# Autodesk Inventor assembly: Stewart Assembly
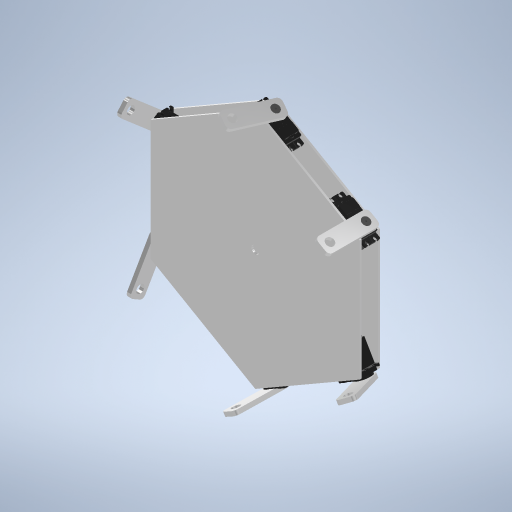
[picture p0: Inventor's stored thumbnail of the model, 512x512]
Saved by Autodesk Inventor 2023 (Build 270158000, 158)
## iProperties
Created: 2022-06-23
Part Number: Stewart Assembly
Document SubType Name: Assembly
Designer: earls
Mass: 1362.34 g
Surface Area: 2982.25 cm^2
Volume: 504.572 cm^3
Density: 2.7 g/cm^3
Author: earls
## Documents named in this file (4)
- F:\Documents\Mechatronic Engineering 5.1\Project\CAD\Stewart Assembly.iam
- F:\Documents\Mechatronic Engineering 5.1\Project\CAD\Bottom plate 2.5mm.ipt
- F:\Documents\Mechatronic Engineering 5.1\Project\CAD\ServoMotor\Servo.ipt
- F:\Documents\Mechatronic Engineering 5.1\Project\CAD\Servo arm.ipt
## Components (14 placed, 3 different names)
1. Bottom plate 2.5mm:1 — Mate:4, Mate:5, Mate:6, Mate:10, Mate:11, Mate:12, Mate:13, Mate:14, Mate:15, Mate:16, Mate:17, Mate:18, Mate:19, Mate:20, Mate:21, Mate:23, Mate:24, Mate:25, Mate:26, Mate:27, Mate:28, Mate:29, Mate:30
2. Servo:2 — Mate:4, Mate:5, Mate:6, Rotational:5
3. Servo:3 — Mate:28, Mate:29, Mate:30, Rotational:6
4. Servo:4 — Mate:10, Mate:11, Mate:12, Rotational:7
5. Servo:5 — Mate:13, Mate:14, Mate:15, Rotational:8
6. Servo:6 — Mate:16, Mate:17, Mate:18, Rotational:4
7. Servo:7 — Mate:19, Mate:20, Mate:21, Mate:22, Rotational:9
8. Bottom plate 2.5mm:2 — Mate:22, Mate:23, Mate:24, Mate:25, Mate:26, Mate:27
9. Servo arm:1 — Rotational:8
10. Servo arm:2 — Rotational:7
11. Servo arm:3 — Rotational:4
12. Servo arm:4 — Rotational:9
13. Servo arm:5 — Rotational:5
14. Servo arm:6 — Rotational:6
## Relationships (30: Mate 24, RevoluteJoint 6)
- Mate:4: Bottom plate 2.5mm:1 ↔ Servo:2
- Mate:5: Bottom plate 2.5mm:1 ↔ Servo:2
- Mate:6: Bottom plate 2.5mm:1 ↔ Servo:2
- Mate:10: Bottom plate 2.5mm:1 ↔ Servo:4
- Mate:11: Bottom plate 2.5mm:1 ↔ Servo:4
- Mate:12: Bottom plate 2.5mm:1 ↔ Servo:4
- Mate:13: Bottom plate 2.5mm:1 ↔ Servo:5
- Mate:14: Bottom plate 2.5mm:1 ↔ Servo:5
- Mate:15: Bottom plate 2.5mm:1 ↔ Servo:5
- Mate:16: Bottom plate 2.5mm:1 ↔ Servo:6
- Mate:17: Bottom plate 2.5mm:1 ↔ Servo:6
- Mate:18: Bottom plate 2.5mm:1 ↔ Servo:6
- Mate:19: Bottom plate 2.5mm:1 ↔ Servo:7
- Mate:20: Bottom plate 2.5mm:1 ↔ Servo:7
- Mate:21: Bottom plate 2.5mm:1 ↔ Servo:7
- Mate:22: Servo:7 ↔ Bottom plate 2.5mm:2
- Mate:23: Bottom plate 2.5mm:1 ↔ Bottom plate 2.5mm:2
- Mate:24: Bottom plate 2.5mm:1 ↔ Bottom plate 2.5mm:2
- Mate:25: Bottom plate 2.5mm:1 ↔ Bottom plate 2.5mm:2
- Mate:26: Bottom plate 2.5mm:1 ↔ Bottom plate 2.5mm:2
- Mate:27: Bottom plate 2.5mm:1 ↔ Bottom plate 2.5mm:2
- Rotational:4 [RevoluteJoint]: Servo:6 ↔ Servo arm:3
- Rotational:5 [RevoluteJoint]: Servo:2 ↔ Servo arm:5
- Mate:28: Bottom plate 2.5mm:1 ↔ Servo:3
- Mate:29: Bottom plate 2.5mm:1 ↔ Servo:3
- Mate:30: Bottom plate 2.5mm:1 ↔ Servo:3
- Rotational:6 [RevoluteJoint]: Servo:3 ↔ Servo arm:6
- Rotational:7 [RevoluteJoint]: Servo:4 ↔ Servo arm:2
- Rotational:8 [RevoluteJoint]: Servo:5 ↔ Servo arm:1
- Rotational:9 [RevoluteJoint]: Servo:7 ↔ Servo arm:4
